# Autodesk Inventor assembly: Final Assembly
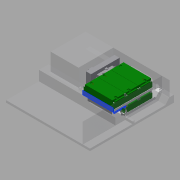
[picture p0: Inventor's stored thumbnail of the model, 180x180]
Saved by Autodesk Inventor 2017 (Build 210142000, 142)
## iProperties
Created: 2022-08-16
Part Number: Final Assembly
Document SubType Name: Assembly
Designer: JTS
Author: JTS
## Documents named in this file (23)
- C:\Users\Windermac\Desktop\MASTER 47 Ah FoMoCo Tray\02 Final Assembly (Tray Mated).iam
- C:\Users\Windermac\Desktop\MASTER 47 Ah FoMoCo Tray\LiBCM003 - Battery Tray\47 Ah FoMoCo Aluminum Tray.ipt
- C:\Users\Windermac\Desktop\MASTER 47 Ah FoMoCo Tray\OEM Parts\Junction Board.ipt
- C:\Users\Windermac\Desktop\MASTER 47 Ah FoMoCo Tray\OEM Parts\MCM.ipt
- C:\Users\Windermac\Desktop\MASTER 47 Ah FoMoCo Tray\Battery Modules\47Ah-FoMoCo.ipt
- C:\Users\Windermac\Desktop\MASTER 47 Ah FoMoCo Tray\LiBCM004 - Battery Rail\Bracket - 5th Module 8982K875.ipt
- C:\Users\Windermac\Desktop\MASTER 47 Ah FoMoCo Tray\Nuts & Bolts\Ring Terminal.ipt
- C:\Users\Windermac\Desktop\MASTER 47 Ah FoMoCo Tray\Final Assembly\AIP\Cable and Harness\Final Assembly.Harness2.iam
- C:\Users\Windermac\Desktop\MASTER 47 Ah FoMoCo Tray\LiBCM PCB\LiBCM Safety Cover - RevC.ipt
- C:\Users\Windermac\Desktop\MASTER 47 Ah FoMoCo Tray\LiBCM PCB\PCB.ipt
- C:\Users\Windermac\Desktop\MASTER 47 Ah FoMoCo Tray\OEM Parts\IMA Bay - Battery Enclosure Interface.ipt
- C:\Users\Windermac\Desktop\MASTER 47 Ah FoMoCo Tray\Nuts & Bolts\Battery Bolt.iam
- C:\Users\Windermac\Desktop\MASTER 47 Ah FoMoCo Tray\Nuts & Bolts\Threaded Standoff.ipt
- C:\Users\Windermac\Desktop\MASTER 47 Ah FoMoCo Tray\Nuts & Bolts\Battery Bolt - Split Washer.iam
- C:\Users\Windermac\Desktop\MASTER 47 Ah FoMoCo Tray\Nuts & Bolts\Washer 0.250in 92141A029.ipt
- C:\Users\Windermac\Desktop\MASTER 47 Ah FoMoCo Tray\Nuts & Bolts\Nut - Hex - 0.250in-20 91845A029.ipt
- C:\Users\Windermac\Desktop\MASTER 47 Ah FoMoCo Tray\Nuts & Bolts\Top Spacer.ipt
- C:\Users\Windermac\Desktop\MASTER 47 Ah FoMoCo Tray\Nuts & Bolts\PEMSERT.ipt
- C:\Users\Windermac\Desktop\MASTER 47 Ah FoMoCo Tray\Grid Chargers\UHP-1500-230.ipt
- C:\Users\Windermac\Desktop\MASTER 47 Ah FoMoCo Tray\Grid Chargers\HLG-480H-C2100B.ipt
- C:\Users\Windermac\Desktop\MASTER 47 Ah FoMoCo Tray\LiBCM005 - Charger Mount\Charger Mount.ipt
- C:\Users\Windermac\Desktop\MASTER 47 Ah FoMoCo Tray\Grid Chargers\HLG-240H-C1050B.ipt
- C:\Users\Windermac\Desktop\MASTER 47 Ah FoMoCo Tray\Nuts & Bolts\Fan.ipt
## Components (64 placed, 22 different names)
1. IMA Bay - Battery Enclosure Interface:1 — Insert:56, Mate:2, Mate:3, Mate:4
2. Junction Board:1 — Insert:11, Insert:12
3. MCM:1 — Insert:9, Insert:10
4. Harness2 [sub-assembly]
5. Washer 0.250in 92141A029:3 — Insert:124
6. Nut - Hex - 0.250in-20 91845A029:5
7. Top Spacer:1 — Insert:125, Insert:126
8. PEMSERT:1 — Insert:129
9. PEMSERT:2 — Insert:130
10. PEMSERT:3 — Insert:131
11. PEMSERT:4 — Insert:132
12. UHP-1500-230:1 — Mate:5, Mate:6, Flush:2, Flush:8, Flush:9
13. HLG-240H-C1050B:1 — Mate:8, Flush:10, Flush:11
14. HLG-480H-C2100B:1 — Mate:7, Flush:8, Flush:9, Flush:10, Flush:11
15. Charger Mount:1 — Flush:5, Flush:6, Mate:8, Insert:133, Insert:134
16. Fan:1 — Insert:133, Insert:134
17. 47 Ah FoMoCo Aluminum Tray:1 — Insert:9, Insert:10, Insert:11, Insert:12, Insert:56, Mate:2, Insert:97, Insert:98, Insert:99, Insert:100, Insert:101, Insert:102, Insert:103, Insert:104, Insert:105, Insert:106, Insert:107, Insert:108, Insert:124
18. LiBCM Safety Cover - RevC:1 — Insert:55, Mate:1, Mate:3, Flush:1, Mate:4
19. PCB:1 — Insert:55, Mate:1
20. Threaded Standoff:1 — Insert:65
21. Threaded Standoff:2 — Insert:70
22. Threaded Standoff:3 — Insert:71
23. Threaded Standoff:4 — Insert:72, Insert:114
24. Threaded Standoff:5 — Insert:69, Insert:113
25. Threaded Standoff:6 — Insert:68, Insert:110
26. Threaded Standoff:7 — Insert:67
27. Threaded Standoff:8 — Insert:66, Insert:109
28. Battery Bolt:1 [sub-assembly] — Insert:102
29. Battery Bolt:2 [sub-assembly] — Insert:101
30. Battery Bolt:3 [sub-assembly] — Insert:99
31. Battery Bolt:4 [sub-assembly] — Insert:98
32. Battery Bolt:5 [sub-assembly] — Insert:100
33. Battery Bolt:6 [sub-assembly] — Insert:104
34. Battery Bolt:7 [sub-assembly] — Insert:103
35. Battery Bolt:8 [sub-assembly] — Insert:97
36. 47Ah-FoMoCo:1 — Insert:41, Insert:43, Tangent:1, Tangent:7, Insert:65, Insert:66, Insert:71, Insert:72, Insert:107, Insert:108
37. 47Ah-FoMoCo:2 — Insert:42, Insert:44, Tangent:3, Tangent:13, Insert:67, Insert:68, Insert:69, Insert:70, Insert:105, Insert:106
38. Bracket - 5th Module 8982K875:1 — Insert:109, Insert:110, Insert:120, Insert:121, Insert:122, Insert:131, Insert:132, Mate:5, Mate:6, Flush:2, Mate:7
39. Bracket - 5th Module 8982K875:2 — Insert:113, Insert:114, Insert:117, Insert:118, Insert:119, Insert:129, Insert:130, Flush:5, Flush:6
40. Battery Bolt:9 [sub-assembly] — Insert:127
41. Battery Bolt:10 [sub-assembly] — Insert:128
42. Battery Bolt - Split Washer:1 [sub-assembly] — Insert:77
43. Battery Bolt - Split Washer:2 [sub-assembly] — Insert:78
44. Battery Bolt - Split Washer:3 [sub-assembly] — Insert:79
45. Battery Bolt - Split Washer:4 [sub-assembly] — Insert:80
46. Battery Bolt - Split Washer:5 [sub-assembly] — Insert:84
47. Battery Bolt - Split Washer:6 [sub-assembly] — Insert:83
48. Battery Bolt - Split Washer:7 [sub-assembly] — Insert:82
49. Battery Bolt - Split Washer:8 [sub-assembly] — Insert:81
50. Battery Bolt - Split Washer:9 [sub-assembly] — Insert:126
51. Battery Bolt - Split Washer:10 [sub-assembly] — Insert:85
52. 47Ah-FoMoCo:3 — Insert:37, Insert:40, Tangent:9, Tangent:12, Flush:1, Insert:79, Insert:80, Insert:81, Insert:82, Insert:121, Insert:122
53. 47Ah-FoMoCo:4 — Insert:36, Insert:39, Tangent:14, Tangent:15, Insert:77, Insert:78, Insert:83, Insert:84, Insert:119, Insert:120
54. 47Ah-FoMoCo:5 — Insert:35, Insert:38, Tangent:16, Tangent:17, Insert:85, Insert:117, Insert:118, Insert:125, Insert:127, Insert:128
55. Ring Terminal:1 — Insert:35, Tangent:16
56. Ring Terminal:2 — Insert:36, Tangent:15
57. Ring Terminal:3 — Insert:37, Tangent:9
58. Ring Terminal:4 — Insert:38, Tangent:17
59. Ring Terminal:5 — Insert:39, Tangent:14
60. Ring Terminal:6 — Insert:40, Tangent:12
61. Ring Terminal:7 — Insert:41, Tangent:1
62. Ring Terminal:8 — Insert:42, Tangent:13
63. Ring Terminal:9 — Insert:43, Tangent:7
64. Ring Terminal:10 — Insert:44, Tangent:3
## Relationships (93: Insert 67, Tangent 10, Mate 8, Flush 8)
- Insert:9: MCM:1 ↔ 47 Ah FoMoCo Aluminum Tray:1
- Insert:10: MCM:1 ↔ 47 Ah FoMoCo Aluminum Tray:1
- Insert:11: Junction Board:1 ↔ 47 Ah FoMoCo Aluminum Tray:1
- Insert:12: Junction Board:1 ↔ 47 Ah FoMoCo Aluminum Tray:1
- Insert:35: 47Ah-FoMoCo:5 ↔ Ring Terminal:1
- Insert:36: 47Ah-FoMoCo:4 ↔ Ring Terminal:2
- Insert:37: 47Ah-FoMoCo:3 ↔ Ring Terminal:3
- Insert:38: 47Ah-FoMoCo:5 ↔ Ring Terminal:4
- Insert:39: 47Ah-FoMoCo:4 ↔ Ring Terminal:5
- Insert:40: 47Ah-FoMoCo:3 ↔ Ring Terminal:6
- Insert:41: 47Ah-FoMoCo:1 ↔ Ring Terminal:7
- Insert:42: 47Ah-FoMoCo:2 ↔ Ring Terminal:8
- Insert:43: 47Ah-FoMoCo:1 ↔ Ring Terminal:9
- Insert:44: 47Ah-FoMoCo:2 ↔ Ring Terminal:10
- Tangent:1 (2 mm): 47Ah-FoMoCo:1 ↔ Ring Terminal:7
- Tangent:3 (4 mm): 47Ah-FoMoCo:2 ↔ Ring Terminal:10
- Tangent:7 (6 mm): 47Ah-FoMoCo:1 ↔ Ring Terminal:9
- Tangent:9 (2 mm): 47Ah-FoMoCo:3 ↔ Ring Terminal:3
- Tangent:12 (2 mm): 47Ah-FoMoCo:3 ↔ Ring Terminal:6
- Tangent:13 (2 mm): 47Ah-FoMoCo:2 ↔ Ring Terminal:8
- Tangent:14 (2 mm): 47Ah-FoMoCo:4 ↔ Ring Terminal:5
- Tangent:15 (2 mm): 47Ah-FoMoCo:4 ↔ Ring Terminal:2
- Tangent:16 (2 mm): 47Ah-FoMoCo:5 ↔ Ring Terminal:1
- Tangent:17 (2 mm): 47Ah-FoMoCo:5 ↔ Ring Terminal:4
- Insert:55 (37 mm): LiBCM Safety Cover - RevC:1 ↔ PCB:1
- Mate:1: LiBCM Safety Cover - RevC:1 ↔ PCB:1
- Insert:56: IMA Bay - Battery Enclosure Interface:1 ↔ 47 Ah FoMoCo Aluminum Tray:1
- Mate:2: IMA Bay - Battery Enclosure Interface:1 ↔ 47 Ah FoMoCo Aluminum Tray:1
- Mate:3 (5 mm): IMA Bay - Battery Enclosure Interface:1 ↔ LiBCM Safety Cover - RevC:1
- Flush:1 (45 mm): LiBCM Safety Cover - RevC:1 ↔ 47Ah-FoMoCo:3
- Mate:4 (31.5 mm): IMA Bay - Battery Enclosure Interface:1 ↔ LiBCM Safety Cover - RevC:1
- Insert:65: Threaded Standoff:1 ↔ 47Ah-FoMoCo:1
- Insert:66: Threaded Standoff:8 ↔ 47Ah-FoMoCo:1
- Insert:67: Threaded Standoff:7 ↔ 47Ah-FoMoCo:2
- Insert:68: Threaded Standoff:6 ↔ 47Ah-FoMoCo:2
- Insert:69: Threaded Standoff:5 ↔ 47Ah-FoMoCo:2
- Insert:70: Threaded Standoff:2 ↔ 47Ah-FoMoCo:2
- Insert:71: Threaded Standoff:3 ↔ 47Ah-FoMoCo:1
- Insert:72: Threaded Standoff:4 ↔ 47Ah-FoMoCo:1
- Insert:77: Battery Bolt - Split Washer:1 ↔ 47Ah-FoMoCo:4
- Insert:78: Battery Bolt - Split Washer:2 ↔ 47Ah-FoMoCo:4
- Insert:79: Battery Bolt - Split Washer:3 ↔ 47Ah-FoMoCo:3
- Insert:80: Battery Bolt - Split Washer:4 ↔ 47Ah-FoMoCo:3
- Insert:81: Battery Bolt - Split Washer:8 ↔ 47Ah-FoMoCo:3
- Insert:82: Battery Bolt - Split Washer:7 ↔ 47Ah-FoMoCo:3
- Insert:83: Battery Bolt - Split Washer:6 ↔ 47Ah-FoMoCo:4
- Insert:84: Battery Bolt - Split Washer:5 ↔ 47Ah-FoMoCo:4
- Insert:85: Battery Bolt - Split Washer:10 ↔ 47Ah-FoMoCo:5
- Insert:97: 47 Ah FoMoCo Aluminum Tray:1 ↔ Battery Bolt:8
- Insert:98: 47 Ah FoMoCo Aluminum Tray:1 ↔ Battery Bolt:4
- Insert:99: 47 Ah FoMoCo Aluminum Tray:1 ↔ Battery Bolt:3
- Insert:100: 47 Ah FoMoCo Aluminum Tray:1 ↔ Battery Bolt:5
- Insert:101: 47 Ah FoMoCo Aluminum Tray:1 ↔ Battery Bolt:2
- Insert:102: 47 Ah FoMoCo Aluminum Tray:1 ↔ Battery Bolt:1
- Insert:103: 47 Ah FoMoCo Aluminum Tray:1 ↔ Battery Bolt:7
- Insert:104: 47 Ah FoMoCo Aluminum Tray:1 ↔ Battery Bolt:6
- Insert:105: 47 Ah FoMoCo Aluminum Tray:1 ↔ 47Ah-FoMoCo:2
- Insert:106: 47 Ah FoMoCo Aluminum Tray:1 ↔ 47Ah-FoMoCo:2
- Insert:107: 47 Ah FoMoCo Aluminum Tray:1 ↔ 47Ah-FoMoCo:1
- Insert:108: 47 Ah FoMoCo Aluminum Tray:1 ↔ 47Ah-FoMoCo:1
- Insert:109: Threaded Standoff:8 ↔ Bracket - 5th Module 8982K875:1
- Insert:110: Threaded Standoff:6 ↔ Bracket - 5th Module 8982K875:1
- Insert:113: Threaded Standoff:5 ↔ Bracket - 5th Module 8982K875:2
- Insert:114: Threaded Standoff:4 ↔ Bracket - 5th Module 8982K875:2
- Insert:117: Bracket - 5th Module 8982K875:2 ↔ 47Ah-FoMoCo:5
- Insert:118: Bracket - 5th Module 8982K875:2 ↔ 47Ah-FoMoCo:5
- Insert:119: Bracket - 5th Module 8982K875:2 ↔ 47Ah-FoMoCo:4
- Insert:120: Bracket - 5th Module 8982K875:1 ↔ 47Ah-FoMoCo:4
- Insert:121: Bracket - 5th Module 8982K875:1 ↔ 47Ah-FoMoCo:3
- Insert:122: Bracket - 5th Module 8982K875:1 ↔ 47Ah-FoMoCo:3
- [Insert]: Washer 0.250in 92141A029:3 ↔ Nut - Hex - 0.250in-20 91845A029:5
- Insert:124: Washer 0.250in 92141A029:3 ↔ 47 Ah FoMoCo Aluminum Tray:1
- Insert:125: Top Spacer:1 ↔ 47Ah-FoMoCo:5
- Insert:126: Top Spacer:1 ↔ Battery Bolt - Split Washer:9
- Insert:127: Battery Bolt:9 ↔ 47Ah-FoMoCo:5
- Insert:128: Battery Bolt:10 ↔ 47Ah-FoMoCo:5
- Insert:129: PEMSERT:1 ↔ Bracket - 5th Module 8982K875:2
- Insert:130: PEMSERT:2 ↔ Bracket - 5th Module 8982K875:2
- Insert:131: PEMSERT:3 ↔ Bracket - 5th Module 8982K875:1
- Insert:132: PEMSERT:4 ↔ Bracket - 5th Module 8982K875:1
- Mate:5: UHP-1500-230:1 ↔ Bracket - 5th Module 8982K875:1
- Mate:6 (1 mm): UHP-1500-230:1 ↔ Bracket - 5th Module 8982K875:1
- Flush:2: UHP-1500-230:1 ↔ Bracket - 5th Module 8982K875:1
- Mate:7: HLG-480H-C2100B:1 ↔ Bracket - 5th Module 8982K875:1
- Flush:5: Charger Mount:1 ↔ Bracket - 5th Module 8982K875:2
- Flush:6: Charger Mount:1 ↔ Bracket - 5th Module 8982K875:2
- Mate:8: HLG-240H-C1050B:1 ↔ Charger Mount:1
- Flush:8: UHP-1500-230:1 ↔ HLG-480H-C2100B:1
- Flush:9: UHP-1500-230:1 ↔ HLG-480H-C2100B:1
- Flush:10: HLG-240H-C1050B:1 ↔ HLG-480H-C2100B:1
- Flush:11: HLG-240H-C1050B:1 ↔ HLG-480H-C2100B:1
- Insert:133: Charger Mount:1 ↔ Fan:1
- Insert:134: Charger Mount:1 ↔ Fan:1
## Named parameters: d147_d115 = 0 mm
